# Autodesk Inventor assembly: 800-BATTERY-PACK
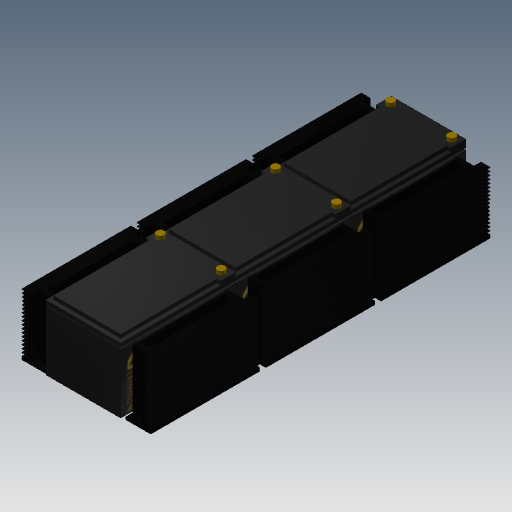
[picture p0: Inventor's stored thumbnail of the model, 512x512]
Saved by Autodesk Inventor 2018.2 (Build 222227000, 227)
## iProperties
Manager: feesmrt
Company: FRANCOR
Part Number: 800-BATTERY-PACK
Project: Rescue Robot
Cost Center: -
Material: Generisch
Document SubType Name: Assembly
Designer: feesmrt
Engineer: feesmrt
Authority: feesmrt
Description: Battery Pack ASM
Stock Number: 800-BATTERY-PACK
Subject: Rescue Robot
Author: feesmrt
Revision Number: 1
Title: Battery Pack ASM
## Documents named in this file (3)
- D:\Programmierung\FRANC0R\CAD\02-Rocker-Bogie-Robot\800-ELECTRONICS\800-BATTERY-PACK.iam
- D:\Programmierung\FRANC0R\CAD\02-Rocker-Bogie-Robot\800-ELECTRONICS\800-10-ELECTRONICS-BATTERY\800-10-ELECTRONICS-BATTERY-12V-12Ah.ipt
- D:\Programmierung\FRANC0R\CAD\02-Rocker-Bogie-Robot\800-ELECTRONICS\800-20-MOTOR-CONTROLLER\800-20-MOTOR-CONTROLLER-BLD-300B.iam
## Components (9 placed, 2 different names)
1. 800-10-ELECTRONICS-BATTERY-12V-12Ah:1 — Fluchtend:1, Fluchtend:2, Fluchtend:3, Fluchtend:4, Passend:1, Passend:2, Fluchtend:5, Passend:7, Fluchtend:12, Fluchtend:13, Passend:10
2. 800-10-ELECTRONICS-BATTERY-12V-12Ah:2 — Fluchtend:1, Fluchtend:2, Passend:2, Passend:5, Fluchtend:7, Fluchtend:8, Passend:8, Passend:11
3. 800-10-ELECTRONICS-BATTERY-12V-12Ah:3 — Fluchtend:3, Fluchtend:4, Passend:1, Passend:3, Passend:4, Fluchtend:9, Fluchtend:10, Passend:6, Fluchtend:11, Passend:9
4. 800-20-MOTOR-CONTROLLER-BLD-300B:1 [sub-assembly] — Passend:3, Fluchtend:5, Fluchtend:6
5. 800-20-MOTOR-CONTROLLER-BLD-300B:2 [sub-assembly] — Passend:4, Fluchtend:9, Fluchtend:10
6. 800-20-MOTOR-CONTROLLER-BLD-300B:3 [sub-assembly] — Passend:5, Fluchtend:7, Fluchtend:8
7. 800-20-MOTOR-CONTROLLER-BLD-300B:4 [sub-assembly] — Passend:7, Fluchtend:12, Passend:10
8. 800-20-MOTOR-CONTROLLER-BLD-300B:5 [sub-assembly] — Passend:6, Fluchtend:11, Passend:9
9. 800-20-MOTOR-CONTROLLER-BLD-300B:6 [sub-assembly] — Passend:8, Fluchtend:13, Passend:11
## Relationships (24: Flush 13, Mate 11)
- Fluchtend:1 [Flush]: 800-10-ELECTRONICS-BATTERY-12V-12Ah:1 ↔ 800-10-ELECTRONICS-BATTERY-12V-12Ah:2
- Fluchtend:2 [Flush]: 800-10-ELECTRONICS-BATTERY-12V-12Ah:1 ↔ 800-10-ELECTRONICS-BATTERY-12V-12Ah:2
- Fluchtend:3 [Flush]: 800-10-ELECTRONICS-BATTERY-12V-12Ah:1 ↔ 800-10-ELECTRONICS-BATTERY-12V-12Ah:3
- Fluchtend:4 [Flush]: 800-10-ELECTRONICS-BATTERY-12V-12Ah:1 ↔ 800-10-ELECTRONICS-BATTERY-12V-12Ah:3
- Passend:1 [Mate]: 800-10-ELECTRONICS-BATTERY-12V-12Ah:1 ↔ 800-10-ELECTRONICS-BATTERY-12V-12Ah:3
- Passend:2 [Mate]: 800-10-ELECTRONICS-BATTERY-12V-12Ah:1 ↔ 800-10-ELECTRONICS-BATTERY-12V-12Ah:2
- Passend:3 [Mate] (2.5 mm): 800-10-ELECTRONICS-BATTERY-12V-12Ah:3 ↔ 800-20-MOTOR-CONTROLLER-BLD-300B:1
- Fluchtend:5 [Flush]: 800-10-ELECTRONICS-BATTERY-12V-12Ah:1 ↔ 800-20-MOTOR-CONTROLLER-BLD-300B:1
- Fluchtend:6 [Flush]: 800-20-MOTOR-CONTROLLER-BLD-300B:1
- Passend:4 [Mate] (2.5 mm): 800-10-ELECTRONICS-BATTERY-12V-12Ah:3 ↔ 800-20-MOTOR-CONTROLLER-BLD-300B:2
- Passend:5 [Mate] (2.5 mm): 800-10-ELECTRONICS-BATTERY-12V-12Ah:2 ↔ 800-20-MOTOR-CONTROLLER-BLD-300B:3
- Fluchtend:7 [Flush]: 800-10-ELECTRONICS-BATTERY-12V-12Ah:2 ↔ 800-20-MOTOR-CONTROLLER-BLD-300B:3
- Fluchtend:8 [Flush]: 800-10-ELECTRONICS-BATTERY-12V-12Ah:2 ↔ 800-20-MOTOR-CONTROLLER-BLD-300B:3
- Fluchtend:9 [Flush]: 800-10-ELECTRONICS-BATTERY-12V-12Ah:3 ↔ 800-20-MOTOR-CONTROLLER-BLD-300B:2
- Fluchtend:10 [Flush]: 800-10-ELECTRONICS-BATTERY-12V-12Ah:3 ↔ 800-20-MOTOR-CONTROLLER-BLD-300B:2
- Passend:6 [Mate] (2.5 mm): 800-10-ELECTRONICS-BATTERY-12V-12Ah:3 ↔ 800-20-MOTOR-CONTROLLER-BLD-300B:5
- Passend:7 [Mate] (2.5 mm): 800-10-ELECTRONICS-BATTERY-12V-12Ah:1 ↔ 800-20-MOTOR-CONTROLLER-BLD-300B:4
- Passend:8 [Mate] (2.5 mm): 800-10-ELECTRONICS-BATTERY-12V-12Ah:2 ↔ 800-20-MOTOR-CONTROLLER-BLD-300B:6
- Fluchtend:11 [Flush]: 800-10-ELECTRONICS-BATTERY-12V-12Ah:3 ↔ 800-20-MOTOR-CONTROLLER-BLD-300B:5
- Fluchtend:12 [Flush]: 800-10-ELECTRONICS-BATTERY-12V-12Ah:1 ↔ 800-20-MOTOR-CONTROLLER-BLD-300B:4
- Fluchtend:13 [Flush]: 800-10-ELECTRONICS-BATTERY-12V-12Ah:1 ↔ 800-20-MOTOR-CONTROLLER-BLD-300B:6
- Passend:9 [Mate]: 800-10-ELECTRONICS-BATTERY-12V-12Ah:3 ↔ 800-20-MOTOR-CONTROLLER-BLD-300B:5
- Passend:10 [Mate]: 800-10-ELECTRONICS-BATTERY-12V-12Ah:1 ↔ 800-20-MOTOR-CONTROLLER-BLD-300B:4
- Passend:11 [Mate]: 800-10-ELECTRONICS-BATTERY-12V-12Ah:2 ↔ 800-20-MOTOR-CONTROLLER-BLD-300B:6
## Named parameters: Battery_Distance = 2.5 mm
